# Autodesk Inventor assembly: Case V3
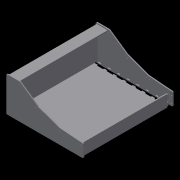
[picture p0: Inventor's stored thumbnail of the model, 180x180]
Saved by Autodesk Inventor 2018 (Build 220112000, 112)
## iProperties
Created: 2017-09-14
Part Number: Case V3
Document SubType Name: Assembly
Designer: gaine
Author: gaine
## Documents named in this file (6)
- C:\Users\gaine\OneDrive\Documents\Eurorack Case\Rev 3\Case V3.iam
- C:\Users\gaine\OneDrive\Documents\Eurorack Case\Rev 3\9U Cheek V3.ipt
- C:\Users\gaine\OneDrive\Documents\Eurorack Case\Rev 3\Top Shelf V3.ipt
- C:\Users\gaine\OneDrive\Documents\Eurorack Case\Rev 3\Back V3.ipt
- C:\Users\gaine\OneDrive\Documents\Eurorack Case\Rev 3\Back 2 V3.ipt
- C:\Users\gaine\OneDrive\Documents\Eurorack Case\Rev 3\Front V3.ipt
## Components (6 placed, 5 different names)
1. 9U Cheek V3:1 — Flush:1, Mate:1, Mate:2, Flush:3, Mate:5, Mate:6, Flush:4, Mate:7, Mate:8, Flush:5, Mate:9, Mate:10
2. 9U Cheek V3:2 — Flush:2, Mate:3, Mate:4
3. Top Shelf V3:1 — Flush:1, Mate:1, Mate:2, Flush:2, Mate:3, Mate:4
4. Back V3:1 — Flush:3, Mate:5, Mate:6
5. Back 2 V3:1 — Flush:4, Mate:7, Mate:8
6. Front V3:1 — Flush:5, Mate:9, Mate:10
## Relationships (15: Mate 10, Flush 5)
- Flush:1: 9U Cheek V3:1 ↔ Top Shelf V3:1
- Mate:1: 9U Cheek V3:1 ↔ Top Shelf V3:1
- Mate:2: 9U Cheek V3:1 ↔ Top Shelf V3:1
- Flush:2: 9U Cheek V3:2 ↔ Top Shelf V3:1
- Mate:3: 9U Cheek V3:2 ↔ Top Shelf V3:1
- Mate:4: 9U Cheek V3:2 ↔ Top Shelf V3:1
- Flush:3: 9U Cheek V3:1 ↔ Back V3:1
- Mate:5: 9U Cheek V3:1 ↔ Back V3:1
- Mate:6: 9U Cheek V3:1 ↔ Back V3:1
- Flush:4: 9U Cheek V3:1 ↔ Back 2 V3:1
- Mate:7: 9U Cheek V3:1 ↔ Back 2 V3:1
- Mate:8: 9U Cheek V3:1 ↔ Back 2 V3:1
- Flush:5: 9U Cheek V3:1 ↔ Front V3:1
- Mate:9: 9U Cheek V3:1 ↔ Front V3:1
- Mate:10: 9U Cheek V3:1 ↔ Front V3:1
